# Autodesk Inventor assembly: Rear_Lower_Arm_V1
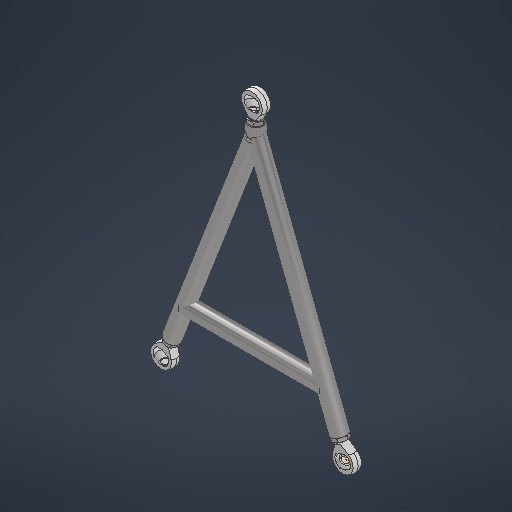
[picture p0: Inventor's stored thumbnail of the model, 512x512]
Saved by Autodesk Inventor 2026.1 (Build 301233000, 233)
## iProperties
Created: 2026-07-13
Part Number: Rear_Lower_Arm_V1
Document SubType Name: Assembly
Designer: share
_SolveAssemblyDoc: Frame Generator Solve Assembly
_Version: 15.0.0
Author: share
## Documents named in this file (5)
- C:\Users\share\OneDrive\Documents\Personal Projects\GOGO Kart\CAD\GOGO_KART_FSAE\Suspension\Suspension Arms\Rear_Lower_Arm_V1\Rear_Lower_Arm_V1.iam
- C:\Users\share\OneDrive\Documents\Personal Projects\GOGO Kart\CAD\GOGO_KART_FSAE\Suspension\Suspension Arms\Arm_Outline_Sketch.ipt
- C:\Users\share\OneDrive\Documents\Personal Projects\GOGO Kart\CAD\GOGO_KART_FSAE\Suspension\Suspension Arms\Rear_Lower_Arm_V1\Rear_Lower_Arm_V1_Frame.iam
- C:\Users\share\OneDrive\Documents\Personal Projects\GOGO Kart\CAD\GOGO_KART_FSAE\Suspension\Suspension Arms\Suspension Rod Ends\5-8 Rod End Assembly.iam
- C:\Users\share\OneDrive\Documents\Inventor\Content Center Files\R2026\en-US\ISO 8675(2)\ISO 8675 - M12 x 1.5 - ISO.ipt
## Components (8 placed, 4 different names)
1. Arm_Outline_Sketch:1 — Flush:1, Flush:2, Flush:3, Mate:1, Mate:3, Mate:4, Mate:5, Mate:7, Mate:8
2. Rear_Lower_Arm_V1_Frame:1 [sub-assembly] — Insert:1, Insert:2, Insert:3
3. 5-8 Rod End Assembly:1 [sub-assembly] — Mate:1, Mate:2, Mate:3
4. 5-8 Rod End Assembly:2 [sub-assembly] — Mate:4, Mate:5, Mate:6
5. 5-8 Rod End Assembly:3 [sub-assembly] — Mate:7, Flush:4, Mate:8
6. ISO 8675 M12 x 1.5:1 — Insert:3
7. ISO 8675 M12 x 1.5:2 — Insert:2
8. ISO 8675 M12 x 1.5:3 — Insert:1
## Relationships (15: Mate 8, Flush 4, Insert 3)
- Flush:1: Arm_Outline_Sketch:1
- Flush:2: Arm_Outline_Sketch:1
- Flush:3: Arm_Outline_Sketch:1
- Mate:1: Arm_Outline_Sketch:1 ↔ 5-8 Rod End Assembly:1
- Mate:2: 5-8 Rod End Assembly:1
- Mate:3: Arm_Outline_Sketch:1 ↔ 5-8 Rod End Assembly:1
- Mate:4: Arm_Outline_Sketch:1 ↔ 5-8 Rod End Assembly:2
- Mate:5: Arm_Outline_Sketch:1 ↔ 5-8 Rod End Assembly:2
- Mate:6: 5-8 Rod End Assembly:2
- Mate:7: Arm_Outline_Sketch:1 ↔ 5-8 Rod End Assembly:3
- Flush:4: 5-8 Rod End Assembly:3
- Mate:8: Arm_Outline_Sketch:1 ↔ 5-8 Rod End Assembly:3
- Insert:1: Rear_Lower_Arm_V1_Frame:1 ↔ ISO 8675 M12 x 1.5:3
- Insert:2: Rear_Lower_Arm_V1_Frame:1 ↔ ISO 8675 M12 x 1.5:2
- Insert:3: Rear_Lower_Arm_V1_Frame:1 ↔ ISO 8675 M12 x 1.5:1
